# Autodesk Inventor assembly: wheel
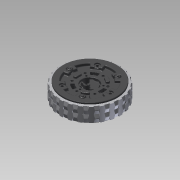
[picture p0: Inventor's stored thumbnail of the model, 180x180]
Saved by Autodesk Inventor 2015 (Build 190159000, 159)
## iProperties
Created: 2015-12-17
Part Number: wheel
Document SubType Name: Assembly
Designer: Daniel
Author: Daniel
## Documents named in this file (3)
- C:\Users\Daniel\Documents\inventor\West Coast Drive\wheel.iam
- C:\Users\Daniel\Documents\inventor\West Coast Drive\217-2588 wheel hub.iam
- C:\Users\Daniel\Documents\inventor\West Coast Drive\217-2859 tire tread.iam
## Components (3 placed, 2 different names)
1. 217-2588 wheel hub:1 [sub-assembly] — Mate:1, Mate:2, Mate:5
2. 217-2859 tire tread:1 [sub-assembly] — Mate:1, Mate:3, Mate:4
3. 217-2859 tire tread:2 [sub-assembly] — Mate:2, Mate:3, Mate:4, Mate:5
## Relationships (5: Mate 5)
- Mate:1: 217-2588 wheel hub:1 ↔ 217-2859 tire tread:1
- Mate:2: 217-2588 wheel hub:1 ↔ 217-2859 tire tread:2
- Mate:3: 217-2859 tire tread:1 ↔ 217-2859 tire tread:2
- Mate:4: 217-2859 tire tread:1 ↔ 217-2859 tire tread:2
- Mate:5: 217-2588 wheel hub:1 ↔ 217-2859 tire tread:2
